# Autodesk Inventor assembly: MKP2 - X Axis
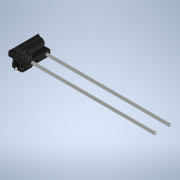
[picture p0: Inventor's stored thumbnail of the model, 180x180]
Saved by Autodesk Inventor 2020.3 (Build 243373010, 373A)
## iProperties
Created: 2021-08-02
Part Number: MKP2 - X Axis
Document SubType Name: Assembly
Designer: Parker
Author: Parker
## Documents named in this file (5)
- D:\Designs\MK3PRO P1\X-Axis\MKP2 - X Axis.iam
- D:\Designs\MK3PRO P1\X-Axis\Teflon T-Nut.ipt
- D:\Designs\MK3PRO P1\X-Axis\MkP2 - X Axis Motor.ipt
- D:\Designs\MK3PRO P1\X-Axis\MKP2 - X-Axis Rod.ipt
- D:\Designs\MK3PRO P1\COMPONENTS\prusa-i3_mk3_r3-1\x-axis-stepper-motor.iam
## Components (5 placed, 4 different names)
1. Teflon T-Nut:1
2. MkP2 - X Axis Motor:1 — Mate:1, Mate:2, Mate:3, Mate:4, Mate:5
3. MKP2 - X-Axis Rod:1
4. MKP2 - X-Axis Rod:2 — Mate:1, Mate:2
5. x-axis-stepper-motor:1 [sub-assembly] — Mate:3, Mate:4, Mate:5
## Relationships (5: Mate 5)
- Mate:1: MkP2 - X Axis Motor:1 ↔ MKP2 - X-Axis Rod:2
- Mate:2: MkP2 - X Axis Motor:1 ↔ MKP2 - X-Axis Rod:2
- Mate:3: MkP2 - X Axis Motor:1 ↔ x-axis-stepper-motor:1
- Mate:4: MkP2 - X Axis Motor:1 ↔ x-axis-stepper-motor:1
- Mate:5: MkP2 - X Axis Motor:1 ↔ x-axis-stepper-motor:1
